# Autodesk Inventor assembly: Arm Yay
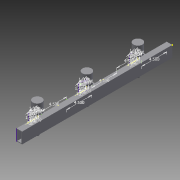
[picture p0: Inventor's stored thumbnail of the model, 180x180]
Saved by Autodesk Inventor 2015 (Build 190159000, 159)
## iProperties
Created: 2015-01-11
Part Number: Arm Yay
Document SubType Name: Assembly
Designer: chapale16
Author: chapale16
## Documents named in this file (3)
- \\lhssvr02\Homedirs\Robotics Club\CAD Model 2015\Game Components\The Tote Collector-Arms\Arm Yay.iam
- \\lhssvr02\Homedirs\Robotics Club\CAD Model 2015\Game Components\The Tote Collector-Arms\P60 Gear Box.ipt
- \\lhssvr02\Homedirs\Robotics Club\CAD Model 2015\Game Components\The Tote Collector-Arms\Arm.ipt
## Components (4 placed, 2 different names)
1. P60 Gear Box:1 — Mate:3
2. P60 Gear Box:2 — Mate:2
3. P60 Gear Box:3 — Mate:1
4. Arm:1 — Mate:1, Mate:2, Mate:3
## Relationships (3: Mate 3)
- Mate:1: P60 Gear Box:3 ↔ Arm:1
- Mate:2: P60 Gear Box:2 ↔ Arm:1
- Mate:3: P60 Gear Box:1 ↔ Arm:1
